# Autodesk Inventor assembly: UpperFrontLink
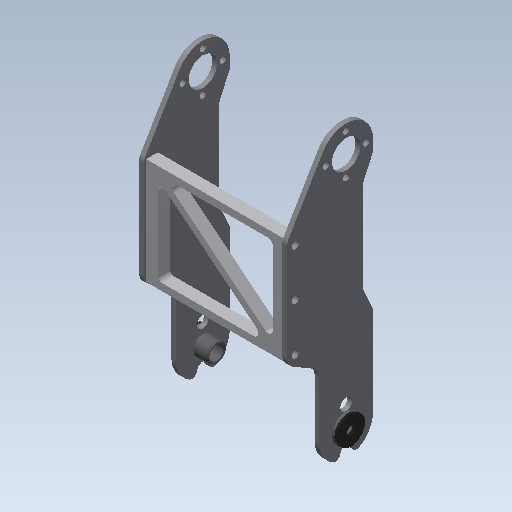
[picture p0: Inventor's stored thumbnail of the model, 512x512]
Saved by Autodesk Inventor 2020 (Build 240168000, 168)
## iProperties
Created: 2016-08-23
Part Number: UpperFrontLink
Material: 一般
Document SubType Name: Assembly
Designer: hiro
Mass: 33.5175 g
Surface Area: 182.778 cm^2
Volume: 15.549 cm^3
Density: 2.15561 g/cm^3
Author: hiro
## Documents named in this file (5)
- C:\Users\Masato\Desktop\最新版\OpenPlatform_ver3_0\下半身\リンク\UpperFrontLink.iam
- C:\Users\Masato\Desktop\最新版\OpenPlatform_ver3_0\下半身\リンク\リンク_ふくらはぎ_サブフレーム_1_1.ipt
- C:\Users\Masato\Desktop\最新版\OpenPlatform_ver3_0\下半身\リンク\リンク_メインフレーム_6_4.ipt
- C:\Users\Masato\Desktop\最新版\OpenPlatform_ver3_0\Ready_Made\80F-0608.ipt
- C:\Users\Masato\Desktop\最新版\OpenPlatform_ver3_0\Ready_Made\UUW-0312-10BH.ipt
## Components (7 placed, 4 different names)
1. リンク_メインフレーム_6_4:1 — 挿入:7, 挿入:8, 挿入:9, 挿入:14
2. リンク_メインフレーム_6_4:2 — 挿入:10, 挿入:11, 挿入:12, 挿入:13
3. リンク_ふくらはぎ_サブフレーム_1_1:1 — 挿入:7, 挿入:8, 挿入:9, 挿入:10, 挿入:11, 挿入:12
4. 80F-0608:1 — 挿入:13, 挿入:16
5. 80F-0608:2 — 挿入:14, 挿入:15
6. UUW-0312-10BH:1 — 挿入:15
7. UUW-0312-10BH:2 — 挿入:16
## Relationships (10: Insert 10)
- 挿入:7 [Insert]: リンク_メインフレーム_6_4:1 ↔ リンク_ふくらはぎ_サブフレーム_1_1:1
- 挿入:8 [Insert]: リンク_メインフレーム_6_4:1 ↔ リンク_ふくらはぎ_サブフレーム_1_1:1
- 挿入:9 [Insert]: リンク_メインフレーム_6_4:1 ↔ リンク_ふくらはぎ_サブフレーム_1_1:1
- 挿入:10 [Insert]: リンク_メインフレーム_6_4:2 ↔ リンク_ふくらはぎ_サブフレーム_1_1:1
- 挿入:11 [Insert]: リンク_メインフレーム_6_4:2 ↔ リンク_ふくらはぎ_サブフレーム_1_1:1
- 挿入:12 [Insert]: リンク_メインフレーム_6_4:2 ↔ リンク_ふくらはぎ_サブフレーム_1_1:1
- 挿入:13 [Insert]: リンク_メインフレーム_6_4:2 ↔ 80F-0608:1
- 挿入:14 [Insert]: リンク_メインフレーム_6_4:1 ↔ 80F-0608:2
- 挿入:15 [Insert]: 80F-0608:2 ↔ UUW-0312-10BH:1
- 挿入:16 [Insert]: 80F-0608:1 ↔ UUW-0312-10BH:2
